# Autodesk Inventor assembly: Assembly2 - Copy_MIR
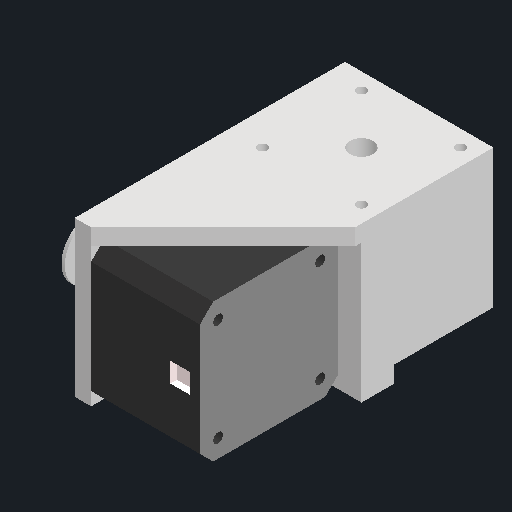
[picture p0: Inventor's stored thumbnail of the model, 512x512]
Saved by Autodesk Inventor 2025.1 (Build 291241000, 241)
## iProperties
Created: 2025-02-02
Part Number: Assembly2 - Copy_MIR
Document SubType Name: Assembly
Designer: jerem
Author: jerem
## Documents named in this file (5)
- C:\Users\jerem\Documents\GitHub\Perovskite-Automated-Synthesis-System\CAD\Gantry\Assembly2 - Copy_MIR.iam
- C:\Users\jerem\Documents\GitHub\Perovskite-Automated-Synthesis-System\CAD\Gantry\X Axis End_MIR1.ipt
- C:\Users\jerem\Documents\GitHub\Perovskite-Automated-Synthesis-System\CAD\Non 3D Printed Parts\Motors and Servos\NEMA17 Stepper Motor_MIR.ipt
- C:\Users\jerem\Documents\GitHub\Perovskite-Automated-Synthesis-System\CAD\Non 3D Printed Parts\Idler_MIR1.ipt
- C:\Users\jerem\Documents\GitHub\Perovskite-Automated-Synthesis-System\CAD\Gantry\otherholderthing_MIR.ipt
## Components (4 placed, 4 different names)
1. X Axis End_MIR1:1 — Flush:1, Mate:14, Mate:13, Mate:16
2. NEMA17 Stepper Motor_MIR:1 — Flush:1, Mate:14, Mate:5, Mate:17, Mate:15
3. Idler_MIR1:1 — Mate:5, Mate:13
4. otherholderthing_MIR:1 — Mate:17, Mate:16, Mate:15
## Relationships (7: Mate 6, Flush 1)
- Flush:1: X Axis End_MIR1:1 ↔ NEMA17 Stepper Motor_MIR:1
- Mate:14: X Axis End_MIR1:1 ↔ NEMA17 Stepper Motor_MIR:1
- Mate:5: NEMA17 Stepper Motor_MIR:1 ↔ Idler_MIR1:1
- Mate:13 (8 mm): X Axis End_MIR1:1 ↔ Idler_MIR1:1
- Mate:17: NEMA17 Stepper Motor_MIR:1 ↔ otherholderthing_MIR:1
- Mate:16: X Axis End_MIR1:1 ↔ otherholderthing_MIR:1
- Mate:15: NEMA17 Stepper Motor_MIR:1 ↔ otherholderthing_MIR:1
